# Autodesk Inventor assembly: inner_glide_carriage_assembly
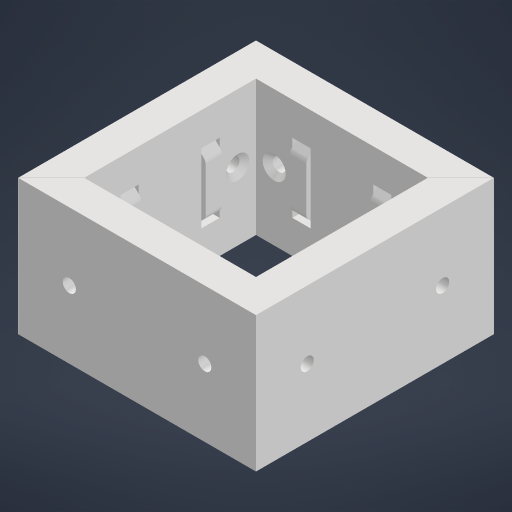
[picture p0: Inventor's stored thumbnail of the model, 512x512]
Saved by Autodesk Inventor 2024 (Build 280153000, 153)
## iProperties
Created: 2023-05-24
Part Number: inner_glide_carriage_assembly
Document SubType Name: Assembly
Designer: aasmu
Author: aasmu
## Documents named in this file (3)
- C:\Users\aasmu\Documents\standing_desk\inner_glide_carriage_assembly.iam
- C:\Users\aasmu\Documents\standing_desk\3_inner_glider_carriage_one_side.ipt
- C:\Users\aasmu\Documents\standing_desk\steal_glide_plate.ipt
## Components (12 placed, 2 different names)
1. 3_inner_glider_carriage_one_side:1 — Rigid:1, Rigid:10, Rigid:11
2. 3_inner_glider_carriage_one_side:2 — Rigid:2, Rigid:3, Rigid:4, Rigid:5
3. 3_inner_glider_carriage_one_side:3 — Rigid:3, Rigid:6, Rigid:7
4. 3_inner_glider_carriage_one_side:4 — Rigid:1, Rigid:2, Rigid:8, Rigid:9
5. steal_glide_plate:1 — Rigid:6
6. steal_glide_plate:2 — Rigid:7
7. steal_glide_plate:3 — Rigid:4
8. steal_glide_plate:4 — Rigid:5
9. steal_glide_plate:5 — Rigid:8
10. steal_glide_plate:6 — Rigid:9
11. steal_glide_plate:7 — Rigid:10
12. steal_glide_plate:8 — Rigid:11
## Relationships (11: WeldJoint 11)
- Rigid:1 [WeldJoint]: 3_inner_glider_carriage_one_side:1 ↔ 3_inner_glider_carriage_one_side:4
- Rigid:2 [WeldJoint]: 3_inner_glider_carriage_one_side:2 ↔ 3_inner_glider_carriage_one_side:4
- Rigid:3 [WeldJoint]: 3_inner_glider_carriage_one_side:2 ↔ 3_inner_glider_carriage_one_side:3
- Rigid:4 [WeldJoint]: 3_inner_glider_carriage_one_side:2 ↔ steal_glide_plate:3
- Rigid:5 [WeldJoint]: 3_inner_glider_carriage_one_side:2 ↔ steal_glide_plate:4
- Rigid:6 [WeldJoint]: 3_inner_glider_carriage_one_side:3 ↔ steal_glide_plate:1
- Rigid:7 [WeldJoint]: 3_inner_glider_carriage_one_side:3 ↔ steal_glide_plate:2
- Rigid:8 [WeldJoint]: 3_inner_glider_carriage_one_side:4 ↔ steal_glide_plate:5
- Rigid:9 [WeldJoint]: 3_inner_glider_carriage_one_side:4 ↔ steal_glide_plate:6
- Rigid:10 [WeldJoint]: 3_inner_glider_carriage_one_side:1 ↔ steal_glide_plate:7
- Rigid:11 [WeldJoint]: 3_inner_glider_carriage_one_side:1 ↔ steal_glide_plate:8
